# Autodesk Inventor assembly: Gehäuse
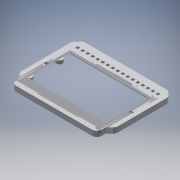
[picture p0: Inventor's stored thumbnail of the model, 180x180]
Saved by Autodesk Inventor 2017 SP1 (Build 210196100, 196)
## iProperties
Part Number: Gehäuse
Material: Generisch
Document SubType Name: Assembly
Designer: aXe
Author: aXe
## Documents named in this file (5)
- C:\Users\aXe\Dropbox\Elektronik\aXe_Dashboard240XL\Gehäuse\Gehäuse.iam
- GehäuseDeckel.iam
- C:\Users\aXe\Dropbox\Elektronik\aXe_Dashboard240XL\Gehäuse\Platine\PCB_SingleLedRow.iam
- C:\Users\aXe\Dropbox\Elektronik\aXe_Dashboard240XL\Gehäuse\Deckel.ipt
- C:\Users\aXe\Dropbox\Elektronik\aXe_Dashboard240XL\Gehäuse\DummyAuschnitt2.ipt
## Components (3 placed, 3 different names)
1. PCB_SingleLedRow:1 [sub-assembly] — Fluchtend:1, Passend:1, Passend:2
2. Deckel:1 — Fluchtend:2, Fluchtend:3, Fluchtend:4
3. DummyAuschnitt2:1 — Fluchtend:1, Passend:1, Passend:2, Fluchtend:2, Fluchtend:3, Fluchtend:4
## Relationships (6: Flush 4, Mate 2)
- Fluchtend:1 [Flush]: PCB_SingleLedRow:1 ↔ DummyAuschnitt2:1
- Passend:1 [Mate] (0.1 mm): PCB_SingleLedRow:1 ↔ DummyAuschnitt2:1
- Passend:2 [Mate] (3.05 mm): PCB_SingleLedRow:1 ↔ DummyAuschnitt2:1
- Fluchtend:2 [Flush]: Deckel:1 ↔ DummyAuschnitt2:1
- Fluchtend:3 [Flush]: Deckel:1 ↔ DummyAuschnitt2:1
- Fluchtend:4 [Flush]: Deckel:1 ↔ DummyAuschnitt2:1
